# Autodesk Inventor assembly: Base Arm Structure
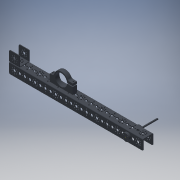
[picture p0: Inventor's stored thumbnail of the model, 180x180]
Saved by Autodesk Inventor 2016 (Build 200138000, 138)
## iProperties
Created: 2015-12-16
Part Number: Base Arm Structure
Document SubType Name: Assembly
Designer: TimB
Author: TimB
## Documents named in this file (6)
- C:\Users\TimB\Documents\GitHub\phi_robotics\3d-models\FTC_Tetrix_KOP_Block_Party\Tim Bloot Designs\JAr JaR Bot\Base Arm Structure.iam
- C:\Users\TimB\Documents\GitHub\phi_robotics\3d-models\FTC_Tetrix_KOP_Block_Party\Tetrix_Kit_FTC\Autodesk Inventor Files\tetrix_c_channel-5.ipt
- C:\Users\TimB\Documents\GitHub\phi_robotics\3d-models\FTC_Tetrix_KOP_Block_Party\Tetrix_Kit_FTC\Autodesk Inventor Files\tetrix_motor_mount-old.ipt
- C:\Users\TimB\Documents\GitHub\phi_robotics\3d-models\FTC_Tetrix_KOP_Block_Party\Tetrix_Kit_FTC\Autodesk Inventor Files\tetrix_c_channel-1.ipt
- C:\Users\TimB\Documents\GitHub\phi_robotics\3d-models\FTC_Tetrix_KOP_Block_Party\Tetrix_Kit_FTC\Autodesk Inventor Files\tetrix_axle_lock.iam
- C:\Users\TimB\Documents\GitHub\phi_robotics\3d-models\FTC_Tetrix_KOP_Block_Party\Tetrix_Kit_FTC\Autodesk Inventor Files\tetrix_axle.ipt
## Components (6 placed, 5 different names)
1. tetrix_c_channel-5:1 — Rigid:1, Rigid:2, Rigid:3, Rigid:4
2. tetrix_motor_mount-old:1 — Rigid:1
3. tetrix_c_channel-1:1 — Rigid:2
4. tetrix_axle_lock:1 [sub-assembly] — Rigid:4, Rigid:5
5. tetrix_axle_lock:2 [sub-assembly] — Rigid:3
6. tetrix_axle:1 — Rigid:5
## Relationships (5: WeldJoint 5)
- Rigid:1 [WeldJoint]: tetrix_c_channel-5:1 ↔ tetrix_motor_mount-old:1
- Rigid:2 [WeldJoint]: tetrix_c_channel-5:1 ↔ tetrix_c_channel-1:1
- Rigid:3 [WeldJoint]: tetrix_c_channel-5:1 ↔ tetrix_axle_lock:2
- Rigid:4 [WeldJoint]: tetrix_c_channel-5:1 ↔ tetrix_axle_lock:1
- Rigid:5 [WeldJoint]: tetrix_axle_lock:1 ↔ tetrix_axle:1
